# Autodesk Inventor assembly: EDMPumpRegionAssembly
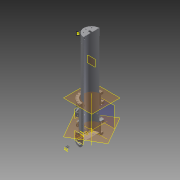
[picture p0: Inventor's stored thumbnail of the model, 180x180]
Saved by Autodesk Inventor 2015 (Build 190159000, 159)
## iProperties
Created: 2014-03-24
Part Number: EDMPumpRegionAssembly
Document SubType Name: Assembly
Designer: jad211
Author: jad211
## Documents named in this file (9)
- C:\CADFiles\EDM Machine\EDM New Pumping Region\EDMPumpRegionAssembly.iam
- C:\CADFiles\EDM Machine\EDM New Pumping Region\NewHorn.ipt
- C:\CADFiles\EDM Machine\EDM New Pumping Region\WG18FLANGECutDown.ipt
- C:\CADFiles\EDM Machine\EDM Middle Shield\EDM Middle shield.ipt
- C:\CADFiles\EDM Machine\EDM Inner Shield\Inner Shield.iam
- C:\CADFiles\EDM Machine\EDM Beamline\Chamber parts\hudson chamber actual size.ipt
- C:\CADFiles\EDM Machine\EDM New Pumping Region\WG18and4SMAFeedthrough.iam
- C:\CADFiles\EDM Machine\EDM New Pumping Region\FlangedWaveguide.iam
- C:\CADFiles\EDM Machine\EDM New Pumping Region\ringLoop.ipt
## Components (11 placed, 8 different names)
1. EDM Middle shield:1 — Mate:8, Flush:11
2. Inner Shield:1 [sub-assembly] — Flush:14, Mate:10, Flush:13, Flush:19
3. hudson chamber actual size:1 — Mate:12, Flush:15, Angle:1, Mate:13
4. NewHorn:1 — Mate:14, Angle:2, Flush:17, Mate:15, Mate:16, Mate:17, Mate:18, Mate:19
5. WG18FLANGECutDown:1 — Flush:17, Mate:15, Mate:16
6. FlangedWaveguide:2 [sub-assembly] — Mate:17, Mate:18, Mate:19, Mate:20, Mate:21, Mate:22
7. WG18and4SMAFeedthrough:1 [sub-assembly] — Mate:20, Mate:21, Mate:22
8. ringLoop:2 — Angle:3, Mate:24, Flush:18
9. ringLoop:3 — Mate:24, Flush:18
10. ringLoop:4
11. ringLoop:5
## Relationships (26: Mate 14, Flush 9, Angle 3)
- Flush:8 (3 mm)
- Mate:8: EDM Middle shield:1
- Flush:11 (158.75 mm): EDM Middle shield:1
- Flush:14 (64.29 mm): Inner Shield:1
- Mate:10: Inner Shield:1
- Flush:13: Inner Shield:1
- Mate:12: hudson chamber actual size:1
- Flush:15: hudson chamber actual size:1
- Flush:16 (-304.8 mm)
- Angle:1 (0 deg): hudson chamber actual size:1
- Mate:13: hudson chamber actual size:1
- Mate:14: NewHorn:1
- Angle:2 (0 deg): NewHorn:1
- Flush:17: NewHorn:1 ↔ WG18FLANGECutDown:1
- Mate:15: NewHorn:1 ↔ WG18FLANGECutDown:1
- Mate:16: NewHorn:1 ↔ WG18FLANGECutDown:1
- Mate:17: NewHorn:1 ↔ FlangedWaveguide:2
- Mate:18: NewHorn:1 ↔ FlangedWaveguide:2
- Mate:19: NewHorn:1 ↔ FlangedWaveguide:2
- Mate:20: FlangedWaveguide:2 ↔ WG18and4SMAFeedthrough:1
- Mate:21: FlangedWaveguide:2 ↔ WG18and4SMAFeedthrough:1
- Mate:22 (30 mm): FlangedWaveguide:2 ↔ WG18and4SMAFeedthrough:1
- Angle:3 (0 deg): ringLoop:2
- Mate:24: ringLoop:2 ↔ ringLoop:3
- Flush:18: ringLoop:2 ↔ ringLoop:3
- Flush:19 (90 mm): Inner Shield:1
